# Autodesk Inventor assembly: RoadBot Pneumatic Module - with Jack - r3
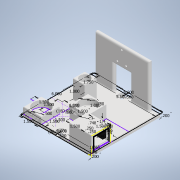
[picture p0: Inventor's stored thumbnail of the model, 180x180]
Saved by Autodesk Inventor 2020 (Build 240168000, 168)
## iProperties
Created: 2022-04-02
Part Number: RoadBot Pneumatic Module - with Jack - r3
Document SubType Name: Assembly
Designer: Beaucage
Author: Beaucage
## Documents named in this file (3)
- V:\AFL\AFL-hardware-devel\AFL-Platform\LoaderGen2\TravelRobotFormFactor\RoadBot Pneumatic Module - with Jack - r3.iam
- V:\AFL\AFL-hardware-devel\AFL-Platform\LoaderGen2\TravelRobotFormFactor\Keystone_Jack_Single_Receptacle (1).ipt
- V:\AFL\AFL-hardware-devel\AFL-Platform\LoaderGen2\TravelRobotFormFactor\RoadBot Pneumatic Module - Base - r2.ipt
## Components (2 placed, 2 different names)
1. RoadBot Pneumatic Module - Base - r2:1 — Mate:1, Mate:2, Flush:1
2. Keystone_Jack_Single_Receptacle (1):1 — Mate:1, Mate:2, Flush:1
## Relationships (3: Mate 2, Flush 1)
- Mate:1: RoadBot Pneumatic Module - Base - r2:1 ↔ Keystone_Jack_Single_Receptacle (1):1
- Mate:2: RoadBot Pneumatic Module - Base - r2:1 ↔ Keystone_Jack_Single_Receptacle (1):1
- Flush:1: RoadBot Pneumatic Module - Base - r2:1 ↔ Keystone_Jack_Single_Receptacle (1):1
